# Autodesk Inventor assembly: 夾爪組合
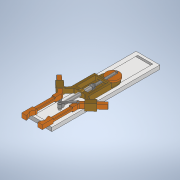
[picture p0: Inventor's stored thumbnail of the model, 180x180]
Saved by Autodesk Inventor 2020 (Build 240168000, 168)
## iProperties
Created: 2021-05-13
Part Number: 夾爪組合
Document SubType Name: Assembly
Designer: User
Author: User
## Documents named in this file (3)
- C:\Users\User\Desktop\stage3-bg1\夾爪組合.iam
- C:\Users\User\Desktop\stage3-bg1\夾爪改.ipt
- C:\Users\User\Desktop\stage3-bg1\滑槽.ipt
## Components (2 placed, 2 different names)
1. 夾爪改:1 — 貼合:1, 貼合:2
2. 滑槽:1 — 貼合:1, 貼合:2
## Relationships (2: Mate 2)
- 貼合:1 [Mate]: 夾爪改:1 ↔ 滑槽:1
- 貼合:2 [Mate]: 夾爪改:1 ↔ 滑槽:1
